# Autodesk Inventor assembly: for_bool
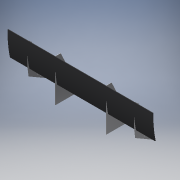
[picture p0: Inventor's stored thumbnail of the model, 180x180]
Saved by Autodesk Inventor 2018.1 (Build 221171000, 171)
## iProperties
Created: 2017-10-22
Part Number: for_bool
Material: 一般
Document SubType Name: Assembly
Designer: ku_sk
Author: ku_sk
## Documents named in this file (4)
- D:\ku_sk\ドキュメント\Inventor\KS-15_Aero_CAD\type4\F-wing\parts\base\for_bool.iam
- D:\ku_sk\ドキュメント\Inventor\KS-15_Aero_CAD\type4\F-wing\parts\base\base.ipt
- D:\ku_sk\ドキュメント\Inventor\KS-15_Aero_CAD\type4\F-wing\parts\stay.ipt
- D:\ku_sk\ドキュメント\Inventor\KS-15_Aero_CAD\type4\F-wing\parts\element_side\parts\stay_middle.ipt
## Components (5 placed, 3 different names)
1. base:1 — メイト:1, メイト:2, メイト:3, メイト:4, メイト:5, フラッシュ:1, フラッシュ:2, メイト:6, フラッシュ:3, フラッシュ:4, フラッシュ:5, フラッシュ:6
2. stay:1 — メイト:2, フラッシュ:1, メイト:7
3. stay:2 — メイト:3, フラッシュ:2, メイト:8
4. stay_middle:1 — メイト:1, メイト:5, フラッシュ:4, メイト:7
5. stay_middle:2 — メイト:4, メイト:6, フラッシュ:3, メイト:8
## Relationships (14: Mate 8, Flush 6)
- メイト:1 [Mate]: base:1 ↔ stay_middle:1
- メイト:2 [Mate]: base:1 ↔ stay:1
- メイト:3 [Mate]: base:1 ↔ stay:2
- メイト:4 [Mate]: base:1 ↔ stay_middle:2
- メイト:5 [Mate]: base:1 ↔ stay_middle:1
- フラッシュ:1 [Flush]: base:1 ↔ stay:1
- フラッシュ:2 [Flush]: base:1 ↔ stay:2
- メイト:6 [Mate]: base:1 ↔ stay_middle:2
- フラッシュ:3 [Flush] (180 mm): base:1 ↔ stay_middle:2
- フラッシュ:4 [Flush] (180 mm): base:1 ↔ stay_middle:1
- メイト:7 [Mate] (260 mm): stay:1 ↔ stay_middle:1
- メイト:8 [Mate] (260 mm): stay:2 ↔ stay_middle:2
- フラッシュ:5 [Flush]: base:1
- フラッシュ:6 [Flush]: base:1
